# Autodesk Inventor assembly: lightweight carrige v2 PROTOX TRY_MIR
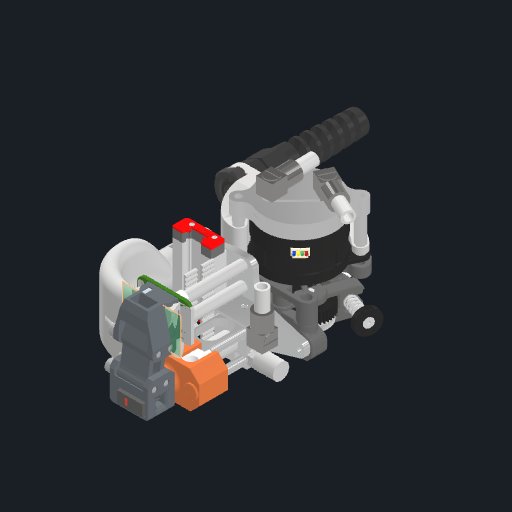
[picture p0: Inventor's stored thumbnail of the model, 512x512]
Saved by Autodesk Inventor 2024.3 (Build 283343010, 343A)
## iProperties
Created: 2024-09-28
Part Number: lightweight carrige v2 PROTOX TRY_MIR
Document SubType Name: Assembly
Designer: MFil
Mass: 257.971 g
Surface Area: 556.316 cm^2
Volume: 46.6137 cm^3
Density: 5.53423 g/cm^3
Author: MFil
## Documents named in this file (29)
- C:\ROBOTYKA\myVORON-tridex\Hotend carriges\lightweight carrige v2 PROTOX TRY_MIR.iam
- C:\ROBOTYKA\myVORON-tridex\Hotend carriges\thin carrige\MGN9H Block_MIR3.ipt
- C:\ROBOTYKA\myVORON-tridex\Hotend carriges\thin carrige\Rocker shaft_MIR3.ipt
- C:\ROBOTYKA\myVORON-tridex\Hotend carriges\thin carrige\Rocker screw BASE_MIR3.iam
- C:\ROBOTYKA\myVORON-tridex\Parts\tridex belt a_CPY 4_MIR3.ipt
- C:\ROBOTYKA\myVORON-tridex\Hotend carriges\parts\filament piece_MIR3.ipt
- C:\ROBOTYKA\myVORON-tridex\Hotend carriges\thin carrige\LDO-36STH20-1004AHG_MIR3.ipt
- C:\ROBOTYKA\myVORON-tridex\Hotend carriges\thin carrige\MR63ZZ (B)_MIR3.ipt
- C:\ROBOTYKA\myVORON-tridex\Hotend carriges\thin carrige\LGX 17T-44T Gear_MIR3.ipt
- C:\ROBOTYKA\myVORON-tridex\Hotend carriges\parts\6mm hose fitting_MIR3.ipt
- C:\ROBOTYKA\myVORON-tridex\Hotend carriges\parts\ptfe filament guide_MIR3.ipt
- C:\ROBOTYKA\myVORON-tridex\Hotend carriges\parts\colle ptfe guide_MIR3.ipt
- C:\ROBOTYKA\myVORON-tridex\Hotend carriges\parts\mounting plate_MIR4.ipt
- C:\ROBOTYKA\myVORON-tridex\Hotend carriges\water hotend v2 assembly_MIR3.iam
- C:\ROBOTYKA\myVORON-tridex\Parts\PG7 Flex Gland\PG7 Flex Gland\PG7 Flex Gland_MIR2.iam
- C:\ROBOTYKA\myVORON-tridex\Hotend carriges\parts\nema 14 heatsink_MIR1.ipt
- C:\ROBOTYKA\myVORON-tridex\Hotend carriges\parts\nema 14 cooler lid_MIR1.ipt
- C:\ROBOTYKA\myVORON-tridex\Hotend carriges\thin carrige\Clicku pcb bottom_MIR.ipt
- C:\ROBOTYKA\myVORON-tridex\Hotend carriges\thin carrige\Part2_MIR.ipt
- C:\ROBOTYKA\myVORON-tridex\Hotend carriges\thin carrige\LGX Hobbed Gear (R)_MIR3.iam
- C:\ROBOTYKA\myVORON-tridex\Extruders\ProtoXtruder_HGX_gears\ProtoXtruder_HGX_gears\Idler_arm_MIR.ipt
- C:\ROBOTYKA\myVORON-tridex\Extruders\ProtoXtruder_HGX_gears\ProtoXtruder_HGX_gears\Back_MIR.ipt
- C:\ROBOTYKA\myVORON-tridex\Hotend carriges\thin carrige\Screw M3x25_MIR3.ipt
- C:\ROBOTYKA\myVORON-tridex\Hotend carriges\parts\pm6m6 fitting dtraight_MIR.ipt
- C:\ROBOTYKA\myVORON-tridex\Hotend carriges\20x5 mm spacer_MIR2.ipt
- C:\ROBOTYKA\myVORON-tridex\Hotend carriges\parts\m3x5 35mm standoff_MIR.ipt
- C:\ROBOTYKA\myVORON-tridex\Hotend carriges\parts\Klicky-00 - RC2 Assemblies\Klicky-00 - RC2 Assemblies\Klicky-00 - RC2 Assemblies_MIR.iam
- C:\ROBOTYKA\myVORON-tridex\step files\ProtoXtruder_HGX_gears\ProtoXtruder_HGX_gears\Front_ECAS04_MIR.ipt
- C:\ROBOTYKA\myVORON-tridex\Parts\umbilical mount_MIR.ipt
## Components (35 placed, 28 different names)
1. MGN9H Block_MIR3:1 — Flush:30, Mate:36, Mate:55, Mate:54, Flush:28
2. Rocker shaft_MIR3:1 — Mate:129
3. Rocker screw BASE_MIR3:1 [sub-assembly] — Mate:131, Mate:130
4. tridex belt a_CPY 4_MIR3:1 — Flush:2, Mate:3, Flush:1
5. tridex belt a_CPY 4_MIR3:2 — Flush:30, Mate:36, Flush:2, Mate:3, Flush:1
6. filament piece_MIR3:1 — Mate:148, Mate:46
7. LDO-36STH20-1004AHG_MIR3:1 — Mate:155, Mate:154, Flush:53, Mate:163, Mate:143, Mate:142, Mate:167, Mate:76, Mate:78
8. MR63ZZ (B)_MIR3:1 — Flush:25, Mate:40
9. LGX 17T-44T Gear_MIR3:1 — Flush:25, Flush:24, Mate:41
10. MR63ZZ (B)_MIR3:2 — Flush:24, Mate:41, Mate:40, Mate:141
11. 6mm hose fitting_MIR3:1 — Mate:161, Mate:70
12. ptfe filament guide_MIR3:1 — Mate:148, Mate:85
13. colle ptfe guide_MIR3:1 — Mate:46
14. mounting plate_MIR4:1 — Mate:55, Mate:54, Flush:28, Mate:174, Mate:173, Mate:84, Flush:115, Mate:165, Flush:114, Mate:166, Mate:164, Mate:71, Mate:72, Mate:73
15. 6mm hose fitting_MIR3:3 — Flush:36
16. 6mm hose fitting_MIR3:4 — Flush:36, Mate:126
17. water hotend v2 assembly_MIR3:1 [sub-assembly] — Mate:174, Mate:173, Mate:161, Mate:85, Mate:84, Mate:145, Flush:120, Flush:118, Flush:117, Mate:169, Mate:69, Mate:70
18. PG7 Flex Gland_MIR2:1 [sub-assembly] — Mate:75, Mate:79
19. nema 14 heatsink_MIR1:1 — Mate:155, Mate:154, Flush:53, Mate:120, Mate:119, Mate:88, Mate:157, Mate:159
20. nema 14 cooler lid_MIR1:1 — Mate:126, Mate:120, Mate:119, Mate:88, Mate:150
21. Clicku pcb bottom_MIR:1
22. Part2_MIR:1 — Flush:115, Flush:119
23. LGX Hobbed Gear (R)_MIR3:1 [sub-assembly] — Flush:110
24. LGX Hobbed Gear (R)_MIR3:2 [sub-assembly] — Flush:110, Flush:109, Mate:128
25. Idler_arm_MIR:1 — Mate:131, Mate:130, Mate:129, Flush:109, Mate:128
26. Back_MIR:1 — Mate:163, Mate:143, Mate:142, Mate:141
27. Screw M3x25_MIR3:1 — Mate:150, Mate:156
28. pm6m6 fitting dtraight_MIR:1 — Mate:145, Mate:69
29. 20x5 mm spacer_MIR2:1 — Mate:157, Mate:156
30. 20x5 mm spacer_MIR2:2 — Mate:167, Mate:159, Mate:77
31. m3x5 35mm standoff_MIR:1 — Mate:165, Flush:114
32. m3x5 35mm standoff_MIR:2 — Mate:166, Mate:164
33. Klicky-00 - RC2 Assemblies_MIR:1 [sub-assembly] — Flush:120, Flush:118, Flush:119, Flush:117, Mate:169
34. Front_ECAS04_MIR:1 — Mate:71, Mate:72, Mate:73
35. umbilical mount_MIR:1 — Mate:75, Mate:76, Mate:77, Mate:78, Mate:79
## Relationships (63: Mate 52, Flush 11)
- Flush:30 (10.831 mm): MGN9H Block_MIR3:1 ↔ tridex belt a_CPY 4_MIR3:2
- Mate:36 (3.3 mm): MGN9H Block_MIR3:1 ↔ tridex belt a_CPY 4_MIR3:2
- Flush:2: tridex belt a_CPY 4_MIR3:1 ↔ tridex belt a_CPY 4_MIR3:2
- Mate:3 (2.5 mm): tridex belt a_CPY 4_MIR3:1 ↔ tridex belt a_CPY 4_MIR3:2
- Flush:1: tridex belt a_CPY 4_MIR3:1 ↔ tridex belt a_CPY 4_MIR3:2
- Flush:25: MR63ZZ (B)_MIR3:1 ↔ LGX 17T-44T Gear_MIR3:1
- Flush:24: LGX 17T-44T Gear_MIR3:1 ↔ MR63ZZ (B)_MIR3:2
- Mate:41: LGX 17T-44T Gear_MIR3:1 ↔ MR63ZZ (B)_MIR3:2
- Mate:40: MR63ZZ (B)_MIR3:1 ↔ MR63ZZ (B)_MIR3:2
- Mate:148: filament piece_MIR3:1 ↔ ptfe filament guide_MIR3:1
- Mate:46: filament piece_MIR3:1 ↔ colle ptfe guide_MIR3:1
- Mate:55: MGN9H Block_MIR3:1 ↔ mounting plate_MIR4:1
- Mate:54: MGN9H Block_MIR3:1 ↔ mounting plate_MIR4:1
- Flush:28 [Mate]: MGN9H Block_MIR3:1 ↔ mounting plate_MIR4:1
- Flush:36: 6mm hose fitting_MIR3:3 ↔ 6mm hose fitting_MIR3:4
- Mate:174: mounting plate_MIR4:1 ↔ water hotend v2 assembly_MIR3:1
- Mate:173: mounting plate_MIR4:1 ↔ water hotend v2 assembly_MIR3:1
- Mate:161: 6mm hose fitting_MIR3:1 ↔ water hotend v2 assembly_MIR3:1
- Mate:85: ptfe filament guide_MIR3:1 ↔ water hotend v2 assembly_MIR3:1
- Mate:84: mounting plate_MIR4:1 ↔ water hotend v2 assembly_MIR3:1
- Mate:155: LDO-36STH20-1004AHG_MIR3:1 ↔ nema 14 heatsink_MIR1:1
- Mate:154: LDO-36STH20-1004AHG_MIR3:1 ↔ nema 14 heatsink_MIR1:1
- Flush:53 [Mate]: LDO-36STH20-1004AHG_MIR3:1 ↔ nema 14 heatsink_MIR1:1
- Mate:126: 6mm hose fitting_MIR3:4 ↔ nema 14 cooler lid_MIR1:1
- Mate:120: nema 14 heatsink_MIR1:1 ↔ nema 14 cooler lid_MIR1:1
- Mate:119: nema 14 heatsink_MIR1:1 ↔ nema 14 cooler lid_MIR1:1
- Mate:88: nema 14 heatsink_MIR1:1 ↔ nema 14 cooler lid_MIR1:1
- Flush:115 [Mate]: mounting plate_MIR4:1 ↔ Part2_MIR:1
- Flush:110: LGX Hobbed Gear (R)_MIR3:1 ↔ LGX Hobbed Gear (R)_MIR3:2
- Mate:131: Rocker screw BASE_MIR3:1 ↔ Idler_arm_MIR:1
- Mate:130: Rocker screw BASE_MIR3:1 ↔ Idler_arm_MIR:1
- Mate:129: Rocker shaft_MIR3:1 ↔ Idler_arm_MIR:1
- Flush:109: LGX Hobbed Gear (R)_MIR3:2 ↔ Idler_arm_MIR:1
- Mate:128: LGX Hobbed Gear (R)_MIR3:2 ↔ Idler_arm_MIR:1
- Mate:163: LDO-36STH20-1004AHG_MIR3:1 ↔ Back_MIR:1
- Mate:143: LDO-36STH20-1004AHG_MIR3:1 ↔ Back_MIR:1
- Mate:142: LDO-36STH20-1004AHG_MIR3:1 ↔ Back_MIR:1
- Mate:141: MR63ZZ (B)_MIR3:2 ↔ Back_MIR:1
- Mate:150: nema 14 cooler lid_MIR1:1 ↔ Screw M3x25_MIR3:1
- Mate:145: water hotend v2 assembly_MIR3:1 ↔ pm6m6 fitting dtraight_MIR:1
- Mate:157: nema 14 heatsink_MIR1:1 ↔ 20x5 mm spacer_MIR2:1
- Mate:156: Screw M3x25_MIR3:1 ↔ 20x5 mm spacer_MIR2:1
- Mate:167: LDO-36STH20-1004AHG_MIR3:1 ↔ 20x5 mm spacer_MIR2:2
- Mate:159: nema 14 heatsink_MIR1:1 ↔ 20x5 mm spacer_MIR2:2
- Mate:165: mounting plate_MIR4:1 ↔ m3x5 35mm standoff_MIR:1
- Flush:114 [Mate]: mounting plate_MIR4:1 ↔ m3x5 35mm standoff_MIR:1
- Mate:166: mounting plate_MIR4:1 ↔ m3x5 35mm standoff_MIR:2
- Mate:164: mounting plate_MIR4:1 ↔ m3x5 35mm standoff_MIR:2
- Flush:120 (3.977 mm): water hotend v2 assembly_MIR3:1 ↔ Klicky-00 - RC2 Assemblies_MIR:1
- Flush:118 (6.474 mm): water hotend v2 assembly_MIR3:1 ↔ Klicky-00 - RC2 Assemblies_MIR:1
- Flush:119 [Mate]: Part2_MIR:1 ↔ Klicky-00 - RC2 Assemblies_MIR:1
- Flush:117: water hotend v2 assembly_MIR3:1 ↔ Klicky-00 - RC2 Assemblies_MIR:1
- Mate:169: water hotend v2 assembly_MIR3:1 ↔ Klicky-00 - RC2 Assemblies_MIR:1
- Mate:69: water hotend v2 assembly_MIR3:1 ↔ pm6m6 fitting dtraight_MIR:1
- Mate:70: 6mm hose fitting_MIR3:1 ↔ water hotend v2 assembly_MIR3:1
- Mate:71: mounting plate_MIR4:1 ↔ Front_ECAS04_MIR:1
- Mate:72: mounting plate_MIR4:1 ↔ Front_ECAS04_MIR:1
- Mate:73: mounting plate_MIR4:1 ↔ Front_ECAS04_MIR:1
- Mate:75: PG7 Flex Gland_MIR2:1 ↔ umbilical mount_MIR:1
- Mate:76: LDO-36STH20-1004AHG_MIR3:1 ↔ umbilical mount_MIR:1
- Mate:77: 20x5 mm spacer_MIR2:2 ↔ umbilical mount_MIR:1
- Mate:78: LDO-36STH20-1004AHG_MIR3:1 ↔ umbilical mount_MIR:1
- Mate:79: PG7 Flex Gland_MIR2:1 ↔ umbilical mount_MIR:1
